# Autodesk Inventor assembly: Assembly2
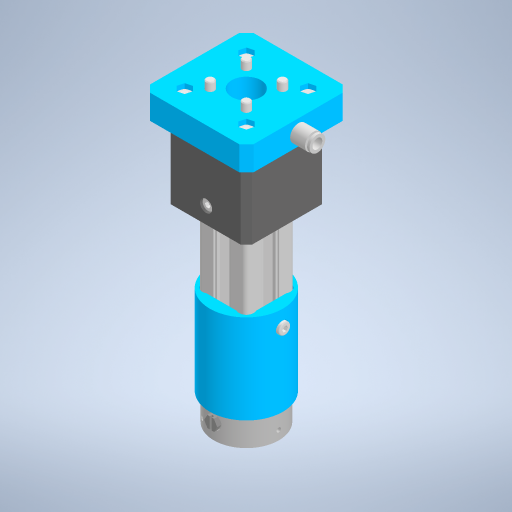
[picture p0: Inventor's stored thumbnail of the model, 512x512]
Saved by Autodesk Inventor 2023 (Build 270158000, 158)
## iProperties
Created: 2022-05-24
Part Number: Assembly2
Document SubType Name: Assembly
Designer: romanp
Author: romanp
## Documents named in this file (14)
- C:\Users\romanp\Downloads\SMC_EE_XT661-4C-X427\Assembly_SMC_EE.iam
- C:\Users\romanp\Downloads\SMC_EE_XT661-4C-X427\Part_Top_b_Blue.ipt
- C:\Users\romanp\Downloads\SMC_EE_XT661-4C-X427\ITEM30x30x100.ipt
- C:\Users\romanp\Downloads\SMC_EE_XT661-4C-X427\M5x25.ipt
- C:\Users\romanp\Downloads\SMC_EE_XT661-4C-X427\M4_nut.ipt
- C:\Users\romanp\Downloads\SMC_EE_XT661-4C-X427\Part_Bottom_Blue.ipt
- C:\Users\romanp\Downloads\SMC_EE_XT661-4C-X427\XT661-4C-X427.iam
- C:\Users\romanp\Downloads\SMC_EE_XT661-4C-X427\KQ2H06-M5N.ipt
- C:\Users\romanp\Downloads\SMC_EE_XT661-4C-X427\M4x25.ipt
- C:\Users\romanp\Downloads\SMC_EE_XT661-4C-X427\M4x20.ipt
- C:\Users\romanp\Downloads\SMC_EE_XT661-4C-X427\KQ2H06-00A.ipt
- C:\Users\romanp\Downloads\SMC_EE_XT661-4C-X427\M4x10.ipt
- C:\Users\romanp\Downloads\SMC_EE_XT661-4C-X427\Part_Middle_Black.ipt
- C:\Users\romanp\Downloads\SMC_EE_XT661-4C-X427\Part_Top_a_Blue.ipt
## Components (30 placed, 13 different names)
1. ITEM30x30x100:4 — Insert:70
2. M5x25:2
3. M4x25:4
4. M4_nut:3
5. M4_nut:4
6. M4_nut:5
7. M4_nut:6
8. M5x25:3
9. M5x25:6
10. M5x25:7
11. M5x25:8
12. KQ2H06-00A:1
13. M4x10:5
14. M4x10:6
15. Part_Bottom_Blue — Insert:57, Insert:58, Insert:60, Insert:61, Insert:62, Insert:63, Insert:64, Insert:65
16. M4x10:7 — Insert:64
17. XT661-4C-X427:3 [sub-assembly] — Insert:57, Insert:58, Insert:59
18. KQ2H06-M5N:3 — Insert:59
19. M4x20:7 — Insert:60
20. M4x20:8 — Insert:63
21. M4x20:9 — Insert:62
22. M4x20:10 — Insert:61
23. M4x10:8 — Insert:65
24. M4x25:5
25. M4x25:6
26. Part_Middle_Black:3 — Insert:70, Insert:71, Insert:73, Insert:74
27. Part_Top_a_Blue:1 — Insert:72
28. Part_Top_b_Blue:5 — Insert:71, Insert:72
29. M4x10:9 — Insert:73
30. M4x10:10 — Insert:74
## Relationships (14: Insert 14)
- Insert:57: Part_Bottom_Blue ↔ XT661-4C-X427:3
- Insert:58: Part_Bottom_Blue ↔ XT661-4C-X427:3
- Insert:59: XT661-4C-X427:3 ↔ KQ2H06-M5N:3
- Insert:60: Part_Bottom_Blue ↔ M4x20:7
- Insert:61: Part_Bottom_Blue ↔ M4x20:10
- Insert:62: Part_Bottom_Blue ↔ M4x20:9
- Insert:63: Part_Bottom_Blue ↔ M4x20:8
- Insert:64: Part_Bottom_Blue ↔ M4x10:7
- Insert:65: Part_Bottom_Blue ↔ M4x10:8
- Insert:70: ITEM30x30x100:4 ↔ Part_Middle_Black:3
- Insert:71: Part_Middle_Black:3 ↔ Part_Top_b_Blue:5
- Insert:72: Part_Top_a_Blue:1 ↔ Part_Top_b_Blue:5
- Insert:73: Part_Middle_Black:3 ↔ M4x10:9
- Insert:74: Part_Middle_Black:3 ↔ M4x10:10
